# Autodesk Inventor assembly: Laser_OnPost
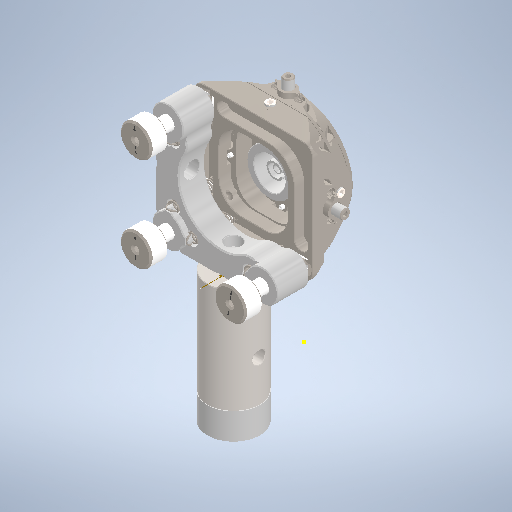
[picture p0: Inventor's stored thumbnail of the model, 512x512]
Saved by Autodesk Inventor 2025.2 (Build 292293000, 293)
## iProperties
Created: 2023-10-20
Part Number: Laser_OnPost
Document SubType Name: Assembly
Designer: S227943
Author: S227943
## Documents named in this file (6)
- C:\Users\monolithic\Documents\GitHub\CAD\Monolith\John\Altair_PowellAndCylindricalBaseplatesCombined_10_16_2025\Assemblies\Subassemblies\Laser_OnPost.iam
- C:\Users\monolithic\Documents\GitHub\CAD\Monolith\John\Altair_PowellBaseplate_SPIM_ASLM_CTASLM\Assembly\SubAssemblies\PLS-P2-1inPost2inTall.ipt
- C:\Users\monolithic\Documents\GitHub\CAD\Monolith\John\Altair_PowellBaseplate_SPIM_ASLM_CTASLM\Assembly\SubAssemblies\PolarisPost_HeightAdjustment_0p5in_smallholesfrom0p79to0p81.ipt
- C:\Users\monolithic\Documents\GitHub\CAD\Monolith\John\Altair_PowellAndCylindricalBaseplatesCombined_10_16_2025\Assemblies\Subassemblies\AD15F-Step\AD15F-Step\AD15F-Step.ipt
- C:\Users\monolithic\Documents\GitHub\CAD\Monolith\John\Altair_PowellBaseplate_SPIM_ASLM_CTASLM\Assembly\SubAssemblies\CFC11A-A.ipt
- C:\Users\monolithic\Documents\GitHub\CAD\Monolith\John\Altair_PowellBaseplate_SPIM_ASLM_CTASLM\Assembly\SubAssemblies\POLARIS-K1XY.ipt
## Components (5 placed, 5 different names)
1. PLS-P2-1inPost2inTall:1 — Mate:3, Mate:4, Mate:14, Mate:15
2. PolarisPost_HeightAdjustment_0p5in_smallholesfrom0p79to0p81:1 — Mate:3, Mate:4
3. AD15F-Step:1 — Mate:9, Mate:10, Mate:11, Mate:13, Flush:1
4. CFC11A-A:1 — Mate:9, Mate:10, Mate:11
5. POLARIS-K1XY:1 — Mate:13, Flush:1, Mate:14, Mate:15
## Relationships (9: Mate 8, Flush 1)
- Mate:3: PLS-P2-1inPost2inTall:1 ↔ PolarisPost_HeightAdjustment_0p5in_smallholesfrom0p79to0p81:1
- Mate:4: PLS-P2-1inPost2inTall:1 ↔ PolarisPost_HeightAdjustment_0p5in_smallholesfrom0p79to0p81:1
- Mate:9: AD15F-Step:1 ↔ CFC11A-A:1
- Mate:10: AD15F-Step:1 ↔ CFC11A-A:1
- Mate:11: AD15F-Step:1 ↔ CFC11A-A:1
- Mate:13: AD15F-Step:1 ↔ POLARIS-K1XY:1
- Flush:1: AD15F-Step:1 ↔ POLARIS-K1XY:1
- Mate:14: PLS-P2-1inPost2inTall:1 ↔ POLARIS-K1XY:1
- Mate:15: PLS-P2-1inPost2inTall:1 ↔ POLARIS-K1XY:1
